# Autodesk Inventor assembly: AM14U Wide Dan's utility proto+shooter
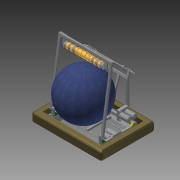
[picture p0: Inventor's stored thumbnail of the model, 180x180]
Saved by Autodesk Inventor 2014 (Build 180170000, 170)
## iProperties
Created: 2014-01-06
Part Number: AM14U Wide Dan's utility proto+shooter
Document SubType Name: Assembly
Designer: robotics
Author: robotics
## Documents named in this file (18)
- C:\Users\pc\Dropbox\Cad 2014 Build Season\Robot 2014\Kitbot\AM14U Wide Dan's utility proto+shooter.iam
- C:\Users\pc\Dropbox\Cad 2014 Build Season\Robot 2014\Imported Components\AM14U Long and AM14U Wide\AM14U Wide Half.iam
- C:\Users\pc\Dropbox\Cad 2014 Build Season\Robot 2014\Kitbot\bumpers.ipt
- C:\Users\pc\Dropbox\Cad 2014 Build Season\Robot 2014\Kitbot\daball.ipt
- C:\Users\pc\Dropbox\CAD\8020\8.ipt
- C:\Users\pc\Dropbox\CAD\4.hole.ipt
- C:\Users\pc\Dropbox\CAD\8020\lg angle.ipt
- C:\Users\pc\Dropbox\CAD\8020\30.ipt
- C:\Users\pc\Dropbox\CAD\24t endcap.ipt
- C:\Users\pc\Dropbox\CAD\lumbrary\CAD Library v2.0\Mechanical\Bearings\AndyMark Bearings\375ID, 1.125OD Shielded Bearing.ipt
- C:\Users\pc\Dropbox\CAD\21 roller.ipt
- C:\Users\pc\Dropbox\CAD\tread.ipt
- C:\Users\pc\Dropbox\CAD\22 shaft.ipt
- C:\Users\pc\Dropbox\CAD\8020\27.ipt
- C:\Users\pc\Dropbox\CAD\3.edit.ipt
- C:\Users\pc\Dropbox\CAD\8020\sm angle.ipt
- C:\Users\pc\Dropbox\CAD\8020\plate1x2.ipt
- C:\Users\pc\Dropbox\Cad 2014 Build Season\Robot 2014\Kitbot\Shooter Prototypes\Driven Shooter.iam
## Components (49 placed, 18 different names)
1. AM14U Wide Half_3 [sub-assembly] — Mate:3, Mate:4, Flush:1, Flush:2, Mate:5, Flush:3, Mate:9, Mate:64, Flush:34
2. AM14U Wide Half_4 [sub-assembly] — Mate:1, Mate:2, Flush:1, Mate:6, Flush:4, Mate:65, Flush:33
3. bumpers:1 — Mate:1, Mate:2, Mate:3, Mate:4, Flush:2, Mate:66, Mate:67
4. daball:1
5. 8:1 — Mate:5, Flush:3, Mate:8, Flush:6, Flush:7, Mate:12, Flush:9
6. 8:2 — Mate:6, Flush:4, Mate:7, Flush:5, Mate:9, Flush:7, Flush:8, Mate:10, Flush:10
7. 4.hole:1 — Flush:8, Mate:10, Mate:11, Mate:14, Mate:15, Flush:10, Flush:11
8. 4.hole:2 — Mate:12, Flush:9, Mate:13, Flush:11, Mate:16, Mate:17
9. lg angle:1 — Mate:7, Flush:5, Mate:11
10. lg angle:2 — Mate:8, Flush:6, Mate:13
11. 4.hole:3 — Mate:14, Mate:15, Flush:12, Mate:18, Flush:13
12. 4.hole:4 — Mate:16, Mate:17, Mate:19, Flush:14, Flush:15
13. 30:1 — Mate:19, Flush:14, Flush:15, Flush:18, Flush:24, Mate:61, Flush:25, Flush:26
14. 30:2 — Flush:12, Mate:18, Flush:13, Mate:49, Flush:16, Flush:17, Flush:29, Mate:62
15. 24t endcap:1
16. 24t endcap:2 — Mate:54
17. 375ID, 1.125OD Shielded Bearing:1 — Mate:55
18. 375ID, 1.125OD Shielded Bearing:2 — Mate:53
19. 21 roller:1 — Mate:54
20. tread:1
21. tread:2
22. tread:3
23. tread:4
24. tread:5
25. tread:6
26. tread:7
27. tread:8
28. tread:9
29. tread:10
30. tread:11
31. tread:12
32. 24 shaft:1 — Mate:52, Flush:21, Flush:22, Mate:53, Mate:55
33. 27:1 — Mate:49, Flush:16, Flush:17, Flush:18, Mate:50, Mate:51, Flush:19, Flush:20, Mate:56, Mate:57, Mate:58, Mate:59, Flush:23, Mate:60, Flush:28, Flush:30, Mate:63, Flush:32
34. 3.edit:1 — Mate:51, Flush:20, Mate:52, Flush:21, Flush:31
35. 3.edit:2 — Mate:50, Flush:19, Flush:22, Flush:27
36. sm angle:1 — Flush:24, Mate:60, Mate:61
37. sm angle:2 — Flush:23, Mate:62, Mate:63
38. plate1x2:1 — Mate:57, Flush:27, Flush:28
39. plate1x2:2 — Mate:58, Flush:31, Flush:32
40. plate1x2:3 — Mate:59, Flush:29, Flush:30
41. plate1x2:4 — Mate:56, Flush:25, Flush:26
42. 8:3 — Mate:64, Flush:34, Mate:66, Mate:69, Mate:70, Flush:36, Flush:37, Mate:77
43. 8:4 — Mate:65, Flush:33, Mate:67, Flush:35, Mate:68, Mate:73, Mate:74, Flush:38, Flush:39
44. 27:2 — Flush:35, Mate:68, Mate:71, Mate:72, Mate:75, Mate:76, Flush:40, Mate:78, Flush:41
45. sm angle:3 — Mate:74, Mate:75, Flush:39
46. sm angle:4 — Mate:73, Mate:76, Flush:38
47. sm angle:5 — Mate:70, Mate:72, Flush:37
48. sm angle:6 — Mate:69, Mate:71, Flush:36, Mate:77
49. Driven Shooter:1 [sub-assembly] — Flush:40, Mate:78, Flush:41
## Relationships (119: Mate 78, Flush 41)
- Mate:1: AM14U Wide Half_4 ↔ bumpers:1
- Mate:2: AM14U Wide Half_4 ↔ bumpers:1
- Mate:3: AM14U Wide Half_3 ↔ bumpers:1
- Mate:4: AM14U Wide Half_3 ↔ bumpers:1
- Flush:1: AM14U Wide Half_3 ↔ AM14U Wide Half_4
- Flush:2 (25.4 mm): AM14U Wide Half_3 ↔ bumpers:1
- Mate:5 (632.079 mm): AM14U Wide Half_3 ↔ 8:1
- Flush:3 (6.35 mm): AM14U Wide Half_3 ↔ 8:1
- Mate:6 (632.079 mm): AM14U Wide Half_4 ↔ 8:2
- Flush:4 (6.35 mm): AM14U Wide Half_4 ↔ 8:2
- Mate:7: 8:2 ↔ lg angle:1
- Flush:5: 8:2 ↔ lg angle:1
- Mate:8: 8:1 ↔ lg angle:2
- Flush:6: 8:1 ↔ lg angle:2
- Mate:9 (25.4 mm): AM14U Wide Half_3 ↔ 8:2
- Flush:7: 8:1 ↔ 8:2
- Flush:8: 8:2 ↔ 4.hole:1
- Mate:10: 8:2 ↔ 4.hole:1
- Mate:11: 4.hole:1 ↔ lg angle:1
- Mate:12: 8:1 ↔ 4.hole:2
- Flush:9: 8:1 ↔ 4.hole:2
- Mate:13: 4.hole:2 ↔ lg angle:2
- Mate:14: 4.hole:1 ↔ 4.hole:3
- Mate:15: 4.hole:1 ↔ 4.hole:3
- Flush:10 (-25.4 mm): 8:2 ↔ 4.hole:1
- Flush:11: 4.hole:1 ↔ 4.hole:2
- Mate:16: 4.hole:2 ↔ 4.hole:4
- Mate:17: 4.hole:2 ↔ 4.hole:4
- Flush:12: 4.hole:3 ↔ 30:2
- Mate:18: 4.hole:3 ↔ 30:2
- Flush:13: 4.hole:3 ↔ 30:2
- Mate:19: 4.hole:4 ↔ 30:1
- Flush:14: 4.hole:4 ↔ 30:1
- Flush:15: 4.hole:4 ↔ 30:1
- [Mate]: 24t endcap:2 ↔ 375ID, 1.125OD Shielded Bearing:2
- [Mate]: 24t endcap:2 ↔ 375ID, 1.125OD Shielded Bearing:2
- [Mate]: 24t endcap:1 ↔ 375ID, 1.125OD Shielded Bearing:1
- [Mate]: 24t endcap:1 ↔ 375ID, 1.125OD Shielded Bearing:1
- [Mate]: 24t endcap:1 ↔ 21 roller:1
- [Mate]: 24t endcap:2 ↔ 21 roller:1
- [Mate]: 21 roller:1 ↔ tread:5
- [Mate]: 21 roller:1 ↔ tread:3
- [Mate]: 21 roller:1 ↔ tread:4
- [Mate]: 21 roller:1 ↔ tread:2
- [Mate]: 21 roller:1 ↔ tread:1
- [Mate]: 21 roller:1 ↔ tread:6
- [Mate]: tread:2 ↔ tread:4
- [Mate] (6.35 mm): tread:1 ↔ tread:2
- [Mate]: tread:1 ↔ tread:3
- [Mate] (6.35 mm): tread:3 ↔ tread:6
- [Mate]: tread:5 ↔ tread:6
- [Mate]: 21 roller:1 ↔ tread:7
- [Mate]: 21 roller:1 ↔ tread:8
- [Mate]: 21 roller:1 ↔ tread:9
- [Mate]: 21 roller:1 ↔ tread:11
- [Mate]: 21 roller:1 ↔ tread:10
- [Mate]: 21 roller:1 ↔ tread:12
- [Mate] (6.35 mm): tread:5 ↔ tread:10
- [Mate] (6.35 mm): tread:4 ↔ tread:9
- [Mate] (33.782 mm): 24t endcap:1 ↔ tread:7
- [Mate] (33.782 mm): tread:7 ↔ tread:8
- [Mate] (33.782 mm): 24t endcap:2 ↔ tread:12
- [Mate] (33.782 mm): tread:11 ↔ tread:12
- Mate:49: 30:2 ↔ 27:1
- Flush:16: 30:2 ↔ 27:1
- Flush:17: 30:2 ↔ 27:1
- Flush:18: 30:1 ↔ 27:1
- Mate:50: 27:1 ↔ 3.edit:2
- Mate:51: 27:1 ↔ 3.edit:1
- Flush:19: 27:1 ↔ 3.edit:2
- Flush:20: 27:1 ↔ 3.edit:1
- Mate:52: 24 shaft:1 ↔ 3.edit:1
- Flush:21: 24 shaft:1 ↔ 3.edit:1
- Flush:22: 24 shaft:1 ↔ 3.edit:2
- Mate:53: 375ID, 1.125OD Shielded Bearing:2 ↔ 24 shaft:1
- Mate:54: 24t endcap:2 ↔ 21 roller:1
- Mate:55: 375ID, 1.125OD Shielded Bearing:1 ↔ 24 shaft:1
- Mate:56: 27:1 ↔ plate1x2:4
- Mate:57: 27:1 ↔ plate1x2:1
- Mate:58: 27:1 ↔ plate1x2:2
- Mate:59: 27:1 ↔ plate1x2:3
- Flush:23: 27:1 ↔ sm angle:2
- Flush:24: 30:1 ↔ sm angle:1
- Mate:60: 27:1 ↔ sm angle:1
- Mate:61: 30:1 ↔ sm angle:1
- Flush:25: 30:1 ↔ plate1x2:4
- Flush:26: 30:1 ↔ plate1x2:4
- Flush:27: 3.edit:2 ↔ plate1x2:1
- Flush:28: 27:1 ↔ plate1x2:1
- Flush:29: 30:2 ↔ plate1x2:3
- Flush:30: 27:1 ↔ plate1x2:3
- Mate:62: 30:2 ↔ sm angle:2
- Mate:63: 27:1 ↔ sm angle:2
- Flush:31: 3.edit:1 ↔ plate1x2:2
- Flush:32: 27:1 ↔ plate1x2:2
- Mate:64: AM14U Wide Half_3 ↔ 8:3
- Mate:65: AM14U Wide Half_4 ↔ 8:4
- Flush:33 (6.35 mm): AM14U Wide Half_4 ↔ 8:4
- Flush:34 (-6.35 mm): AM14U Wide Half_3 ↔ 8:3
- Mate:66 (25.4 mm): bumpers:1 ↔ 8:3
- Mate:67 (25.4 mm): bumpers:1 ↔ 8:4
- Flush:35: 8:4 ↔ 27:2
- Mate:68: 8:4 ↔ 27:2
- Mate:69: 8:3 ↔ sm angle:6
- Mate:70: 8:3 ↔ sm angle:5
- Mate:71: 27:2 ↔ sm angle:6
- Mate:72: 27:2 ↔ sm angle:5
- Flush:36: 8:3 ↔ sm angle:6
- Flush:37: 8:3 ↔ sm angle:5
- Mate:73: 8:4 ↔ sm angle:4
- Mate:74: 8:4 ↔ sm angle:3
- Mate:75: 27:2 ↔ sm angle:3
- Mate:76: 27:2 ↔ sm angle:4
- Flush:38: 8:4 ↔ sm angle:4
- Flush:39: 8:4 ↔ sm angle:3
- Mate:77: 8:3 ↔ sm angle:6
- Flush:40: 27:2 ↔ Driven Shooter:1
- Mate:78: 27:2 ↔ Driven Shooter:1
- Flush:41 (-79.375 mm): 27:2 ↔ Driven Shooter:1
## Named parameters: d95_d38 = 0 mm, d97_d41 = 0 mm, d98_d42 = 0 mm, d99_d36 = 0 mm
